# Autodesk Inventor assembly: wheel_axle
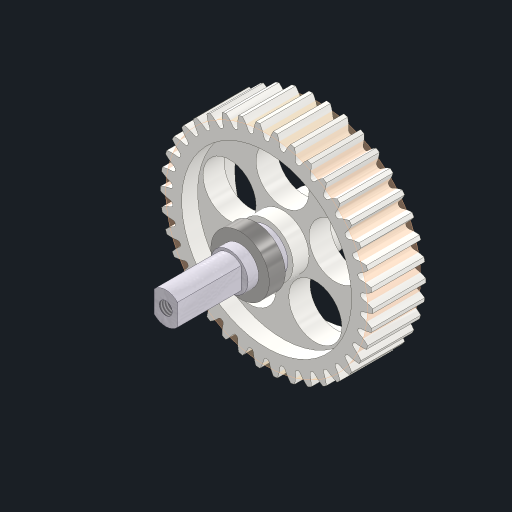
[picture p0: Inventor's stored thumbnail of the model, 512x512]
Saved by Autodesk Inventor 2023 (Build 270158000, 158)
## iProperties
Created: 2024-04-09
Part Number: wheel_axle
Document SubType Name: Assembly
Designer: szymo
Mass: 22 g
Surface Area: 66.799 cm^2
Volume: 6.27657 cm^3
Density: 3.5051 g/cm^3
Author: szymo
## Documents named in this file (5)
- D:\roboilo\robots\codename wafel - australia\3d_parts\rev4\wheel_axle.iam
- D:\roboilo\robots\codename wafel - australia\3d_parts\rev4\MegaSumo kola zebate 38.ipt
- D:\roboilo\robots\codename wafel - australia\3d_parts\rev4\wal_kola.ipt
- D:\roboilo\robots\codename wafel - australia\3d_parts\rev4\small_bearing.ipt
- D:\roboilo\robots\codename wafel - australia\3d_parts\rev4\big_bearing.ipt
## Components (4 placed, 4 different names)
1. wal_kola:1 — Rotational:1, Mate:3, Mate:4, Mate:5, Mate:6
2. MegaSumo kola zebate 38:1 — Rotational:1
3. small_bearing:1 — Mate:3, Mate:4
4. big_bearing:1 — Mate:5, Mate:6
## Relationships (5: Mate 4, RevoluteJoint 1)
- Rotational:1 [RevoluteJoint]: wal_kola:1 ↔ MegaSumo kola zebate 38:1
- Mate:3: wal_kola:1 ↔ small_bearing:1
- Mate:4: wal_kola:1 ↔ small_bearing:1
- Mate:5: wal_kola:1 ↔ big_bearing:1
- Mate:6: wal_kola:1 ↔ big_bearing:1
